# Autodesk Inventor assembly: Omni-Wheel_Assembly
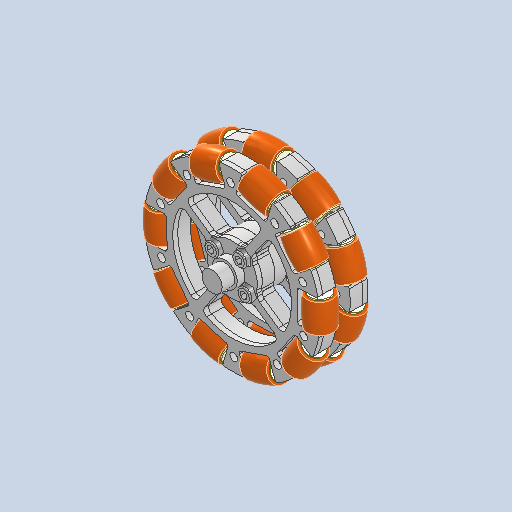
[picture p0: Inventor's stored thumbnail of the model, 512x512]
Saved by Autodesk Inventor 2025 (Build 290162000, 162)
## iProperties
Created: 2024-06-26
Part Number: Omni-Wheel_Assembly
Document SubType Name: Assembly
Designer: 8326d
Author: 8326d
## Documents named in this file (5)
- C:\Users\8326d\Documents\hobby\CAD\General-Purpose-Robot\Omni-Wheel\Omni-Wheel_Assembly.iam
- C:\Users\8326d\Documents\hobby\CAD\General-Purpose-Robot\Omni-Wheel\Omni-Wheel_r1.iam
- C:\Users\8326d\Documents\hobby\CAD\General-Purpose-Robot\Omni-Wheel\AR20.0_inside-shaft.ipt
- C:\Users\8326d\Documents\hobby\CAD\General-Purpose-Robot\Screws\Bolts\M3-CapScrew-L20\M3-CapScrew-L20.ipt
- C:\Users\8326d\Documents\hobby\CAD\General-Purpose-Robot\Screws\Nuts\M3-HexNut-type2\M3-HexNut-type2.ipt
## Components (11 placed, 4 different names)
1. Omni-Wheel_r1:1 [sub-assembly] — 挿入:3, 挿入:4, 挿入:5, 挿入:6, 挿入:7, 挿入:8, 角度:1, 角度:2, 角度:3, 角度:4
2. Omni-Wheel_r1:2 [sub-assembly] — 挿入:1, 挿入:2, 挿入:9, 挿入:10, 挿入:11, 挿入:12
3. AR20.0_inside-shaft:1 — メイト:1, フラッシュ:1, 挿入:1, 挿入:2, 挿入:3, 挿入:4
4. M3-CapScrew-L20:1 — 挿入:9
5. M3-CapScrew-L20:2 — 挿入:10
6. M3-CapScrew-L20:3 — 挿入:11
7. M3-CapScrew-L20:4 — 挿入:12
8. M3-HexNut-type2:1 — 挿入:5, 角度:1
9. M3-HexNut-type2:2 — 挿入:6, 角度:2
10. M3-HexNut-type2:3 — 挿入:7, 角度:3
11. M3-HexNut-type2:4 — 挿入:8, 角度:4
## Relationships (18: Insert 12, Angle 4, Mate 1, Flush 1)
- メイト:1 [Mate]: AR20.0_inside-shaft:1
- フラッシュ:1 [Flush]: AR20.0_inside-shaft:1
- 挿入:1 [Insert]: Omni-Wheel_r1:2 ↔ AR20.0_inside-shaft:1
- 挿入:2 [Insert]: Omni-Wheel_r1:2 ↔ AR20.0_inside-shaft:1
- 挿入:3 [Insert]: Omni-Wheel_r1:1 ↔ AR20.0_inside-shaft:1
- 挿入:4 [Insert]: Omni-Wheel_r1:1 ↔ AR20.0_inside-shaft:1
- 挿入:5 [Insert]: Omni-Wheel_r1:1 ↔ M3-HexNut-type2:1
- 挿入:6 [Insert]: Omni-Wheel_r1:1 ↔ M3-HexNut-type2:2
- 挿入:7 [Insert]: Omni-Wheel_r1:1 ↔ M3-HexNut-type2:3
- 挿入:8 [Insert]: Omni-Wheel_r1:1 ↔ M3-HexNut-type2:4
- 角度:1 [Angle] (0 deg): Omni-Wheel_r1:1 ↔ M3-HexNut-type2:1
- 角度:2 [Angle] (0 deg): Omni-Wheel_r1:1 ↔ M3-HexNut-type2:2
- 角度:3 [Angle] (0 deg): Omni-Wheel_r1:1 ↔ M3-HexNut-type2:3
- 角度:4 [Angle] (0 deg): Omni-Wheel_r1:1 ↔ M3-HexNut-type2:4
- 挿入:9 [Insert]: Omni-Wheel_r1:2 ↔ M3-CapScrew-L20:1
- 挿入:10 [Insert]: Omni-Wheel_r1:2 ↔ M3-CapScrew-L20:2
- 挿入:11 [Insert]: Omni-Wheel_r1:2 ↔ M3-CapScrew-L20:3
- 挿入:12 [Insert]: Omni-Wheel_r1:2 ↔ M3-CapScrew-L20:4
